# Autodesk Inventor assembly: Sorting Assembly
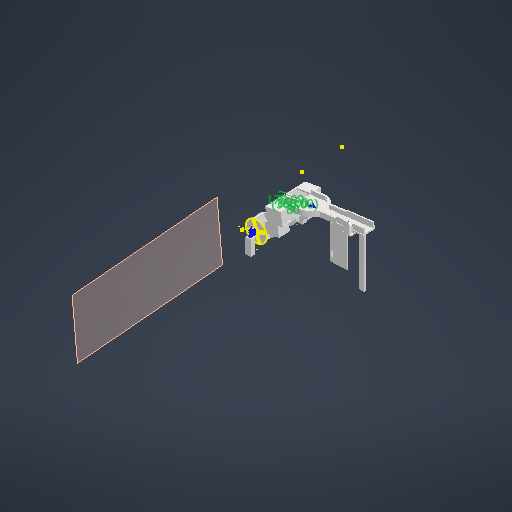
[picture p0: Inventor's stored thumbnail of the model, 512x512]
Saved by Autodesk Inventor 2026.2 (Build 302298000, 298)
## iProperties
Created: 2026-02-23
Part Number: Sorting Assembly
Document SubType Name: Assembly
Designer: danda
Author: danda
## Documents named in this file (2)
- C:\Users\danda\BOM-project\Project\CAD\sorting\Sorting Assembly.iam
- C:\Users\danda\BOM-project\Project\CAD\sorting\Assembly2.iam
## Components (1 placed, 1 different names)
1. Assembly2:1 [sub-assembly] — Mate:1
## Relationships (1: Mate 1)
- Mate:1: Assembly2:1
